# Autodesk Inventor assembly: Forearm2
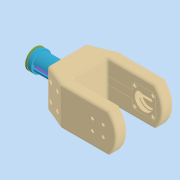
[picture p0: Inventor's stored thumbnail of the model, 180x180]
Saved by Autodesk Inventor 2021 (Build 250183000, 183)
## iProperties
Created: 2020-03-07
Part Number: Forearm2
Document SubType Name: Assembly
Designer: JochenAlt
Author: JochenAlt
## Documents named in this file (4)
- C:\Users\Jochen Alt\Documents\Daten\Projects\MiniBot\CAD\Forearm.iam
- C:\Users\Jochen Alt\Documents\Daten\Projects\MiniBot\CAD\Forearm.ipt
- C:\Users\Jochen Alt\Documents\Daten\Projects\MiniBot\CAD\ForearmShaft.ipt
- C:\Users\Jochen Alt\Documents\Daten\Projects\MiniBot\CAD\extern\bearings\25x32x4\W 61705-2RS1.iam
## Components (4 placed, 3 different names)
1. Forearm:1 — Passend:2, Passend:7
2. ForearmShaft:1 — Passend:2, Passend:3, Passend:4, Passend:5, Passend:6, Passend:7
3. W 61705-2RS1:1 [sub-assembly] — Passend:3, Passend:5
4. W 61705-2RS1:2 [sub-assembly] — Passend:4, Passend:6
## Relationships (6: Mate 6)
- Passend:2 [Mate]: Forearm:1 ↔ ForearmShaft:1
- Passend:3 [Mate]: ForearmShaft:1 ↔ W 61705-2RS1:1
- Passend:4 [Mate]: ForearmShaft:1 ↔ W 61705-2RS1:2
- Passend:5 [Mate]: ForearmShaft:1 ↔ W 61705-2RS1:1
- Passend:6 [Mate]: ForearmShaft:1 ↔ W 61705-2RS1:2
- Passend:7 [Mate]: Forearm:1 ↔ ForearmShaft:1
